# Autodesk Inventor assembly: Rack-Assembly
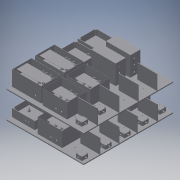
[picture p0: Inventor's stored thumbnail of the model, 180x180]
Saved by Autodesk Inventor 2018 (Build 220112000, 112)
## iProperties
Created: 2018-04-30
Part Number: Rack-Assembly
Document SubType Name: Assembly
Designer: bbramman
Author: bbramman
## Documents named in this file (11)
- C:\Users\bbramman\OneDrive\Documents\Trapped Ion Research (Grad)\Electronics\pll-evalboard-synthesizer\Box CAD\Rack-Assembly.iam
- C:\Users\bbramman\OneDrive\Documents\Trapped Ion Research (Grad)\Electronics\pll-evalboard-synthesizer\Box CAD\Drawer.ipt
- C:\Users\bbramman\OneDrive\Documents\Trapped Ion Research (Grad)\Electronics\pll-evalboard-synthesizer\Box CAD\ADF4355-Enclosure.iam
- C:\Users\bbramman\OneDrive\Documents\Trapped Ion Research (Grad)\Electronics\pll-evalboard-synthesizer\Box CAD\ADF41020-Enclosure.iam
- C:\Users\bbramman\OneDrive\Documents\Trapped Ion Research (Grad)\Electronics\pll-evalboard-synthesizer\Box CAD\ADL5534-Enclosure.iam
- C:\Users\bbramman\OneDrive\Documents\Trapped Ion Research (Grad)\Electronics\pll-evalboard-synthesizer\Box CAD\ADF4360-Enclosure.iam
- C:\Users\bbramman\OneDrive\Documents\Trapped Ion Research (Grad)\Electronics\pll-evalboard-synthesizer\Box CAD\4xSplitter-Enclosure.iam
- C:\Users\bbramman\OneDrive\Documents\Trapped Ion Research (Grad)\Electronics\pll-evalboard-synthesizer\Box CAD\PE4312-Enclosure.iam
- C:\Users\bbramman\OneDrive\Documents\Trapped Ion Research (Grad)\Electronics\pll-evalboard-synthesizer\Box CAD\3xCombiner-Enclosure.iam
- C:\Users\bbramman\OneDrive\Documents\Trapped Ion Research (Grad)\Electronics\pll-evalboard-synthesizer\Box CAD\Shield.ipt
- C:\Users\bbramman\OneDrive\Documents\Trapped Ion Research (Grad)\Electronics\pll-evalboard-synthesizer\Box CAD\ZFSWHA-1-20+_Switch.ipt
## Components (31 placed, 10 different names)
1. Drawer:1 — Mate:6, Mate:8, Mate:9, Mate:11, Mate:12, Mate:13, Mate:16, Flush:1, Flush:2, Mate:23, Mate:24, Mate:25, Mate:26, Flush:3, Flush:4, Flush:5, Flush:6, Mate:36, Mate:37, Mate:38, Mate:39
2. ADF41020-Enclosure:1 [sub-assembly] — Mate:6
3. PE4312-Enclosure:1 [sub-assembly] — Mate:9
4. ADF4355-Enclosure:1 [sub-assembly] — Mate:8
5. PE4312-Enclosure:3 [sub-assembly] — Mate:13
6. ADF4355-Enclosure:2 [sub-assembly] — Mate:11
7. ADF41020-Enclosure:3 [sub-assembly] — Mate:12
8. 3xCombiner-Enclosure:1 [sub-assembly] — Mate:38
9. 3xCombiner-Enclosure:2 [sub-assembly] — Mate:39
10. Drawer:2 — Mate:16, Flush:1, Flush:2, Mate:17, Mate:18, Mate:19, Mate:21, Mate:22, Mate:27, Mate:28, Mate:29, Mate:30, Flush:7, Flush:8, Flush:9, Flush:10, Mate:31, Mate:32, Mate:33, Mate:34, Mate:35, Mate:40
11. ADF4355-Enclosure:3 [sub-assembly] — Mate:17
12. ADF4360-Enclosure:1 [sub-assembly] — Mate:18
13. PE4312-Enclosure:4 [sub-assembly] — Mate:19
14. 4xSplitter-Enclosure:1 [sub-assembly] — Mate:40
15. ADL5534-Enclosure:1 [sub-assembly] — Mate:21
16. PE4312-Enclosure:5 [sub-assembly] — Mate:22
17. Shield:1 — Mate:26, Flush:6
18. Shield:2 — Mate:25, Flush:5
19. Shield:3 — Mate:24, Flush:4
20. Shield:4 — Mate:23, Flush:3
21. Shield:5 — Mate:27, Flush:10
22. Shield:6 — Mate:28, Flush:9
23. Shield:7 — Mate:29, Flush:8
24. Shield:8 — Mate:30, Flush:7
25. ZFSWHA-1-20+_Switch:1 — Mate:31
26. ZFSWHA-1-20+_Switch:2 — Mate:33
27. ZFSWHA-1-20+_Switch:3 — Mate:32
28. ZFSWHA-1-20+_Switch:4 — Mate:34
29. ZFSWHA-1-20+_Switch:5 — Mate:35
30. ZFSWHA-1-20+_Switch:6 — Mate:36
31. ZFSWHA-1-20+_Switch:7 — Mate:37
## Relationships (40: Mate 30, Flush 10)
- Mate:6: Drawer:1 ↔ ADF41020-Enclosure:1
- Mate:8: Drawer:1 ↔ ADF4355-Enclosure:1
- Mate:9: Drawer:1 ↔ PE4312-Enclosure:1
- Mate:11: Drawer:1 ↔ ADF4355-Enclosure:2
- Mate:12: Drawer:1 ↔ ADF41020-Enclosure:3
- Mate:13: Drawer:1 ↔ PE4312-Enclosure:3
- Mate:16 (133.35 mm): Drawer:1 ↔ Drawer:2
- Flush:1: Drawer:1 ↔ Drawer:2
- Flush:2: Drawer:1 ↔ Drawer:2
- Mate:17: Drawer:2 ↔ ADF4355-Enclosure:3
- Mate:18: Drawer:2 ↔ ADF4360-Enclosure:1
- Mate:19: Drawer:2 ↔ PE4312-Enclosure:4
- Mate:21: Drawer:2 ↔ ADL5534-Enclosure:1
- Mate:22: Drawer:2 ↔ PE4312-Enclosure:5
- Mate:23: Drawer:1 ↔ Shield:4
- Mate:24: Drawer:1 ↔ Shield:3
- Mate:25: Drawer:1 ↔ Shield:2
- Mate:26: Drawer:1 ↔ Shield:1
- Flush:3: Drawer:1 ↔ Shield:4
- Flush:4: Drawer:1 ↔ Shield:3
- Flush:5: Drawer:1 ↔ Shield:2
- Flush:6: Drawer:1 ↔ Shield:1
- Mate:27: Drawer:2 ↔ Shield:5
- Mate:28: Drawer:2 ↔ Shield:6
- Mate:29: Drawer:2 ↔ Shield:7
- Mate:30: Drawer:2 ↔ Shield:8
- Flush:7: Drawer:2 ↔ Shield:8
- Flush:8: Drawer:2 ↔ Shield:7
- Flush:9: Drawer:2 ↔ Shield:6
- Flush:10: Drawer:2 ↔ Shield:5
- Mate:31: Drawer:2 ↔ ZFSWHA-1-20+_Switch:1
- Mate:32: Drawer:2 ↔ ZFSWHA-1-20+_Switch:3
- Mate:33: Drawer:2 ↔ ZFSWHA-1-20+_Switch:2
- Mate:34: Drawer:2 ↔ ZFSWHA-1-20+_Switch:4
- Mate:35: Drawer:2 ↔ ZFSWHA-1-20+_Switch:5
- Mate:36: Drawer:1 ↔ ZFSWHA-1-20+_Switch:6
- Mate:37: Drawer:1 ↔ ZFSWHA-1-20+_Switch:7
- Mate:38: Drawer:1 ↔ 3xCombiner-Enclosure:1
- Mate:39: Drawer:1 ↔ 3xCombiner-Enclosure:2
- Mate:40: Drawer:2 ↔ 4xSplitter-Enclosure:1
